# Autodesk Inventor assembly: Door Moulding Assembled
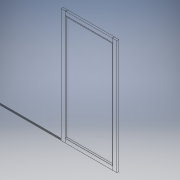
[picture p0: Inventor's stored thumbnail of the model, 180x180]
Saved by Autodesk Inventor 2016 (Build 200138000, 138)
## iProperties
Created: 2017-11-05
Part Number: Door Moulding Assembled
Document SubType Name: Assembly
Designer: mathaetaes
Author: mathaetaes
## Documents named in this file (4)
- E:\Projects\3D Printer\printer projects\My Designs\Bar Cabinet 2.20.2018\Door Moulding Assembled.iam
- E:\Projects\3D Printer\printer projects\My Designs\Bar Cabinet 2.20.2018\Cabinet Moulding Long.ipt
- E:\Projects\3D Printer\printer projects\My Designs\Bar Cabinet 2.20.2018\Door moulding slide-in panel.ipt
- E:\Projects\3D Printer\printer projects\My Designs\Bar Cabinet 2.20.2018\Cabinet Moulding Short.ipt
## Components (5 placed, 3 different names)
1. Cabinet Moulding Long:1 — Mate:2, Mate:3, Flush:2, Flush:4, Flush:5, Mate:6, Flush:6, Mate:7, Mate:8
2. Cabinet Moulding Long:2 — Mate:1, Mate:4, Flush:1, Flush:3
3. Door moulding slide-in panel:1 — Mate:5, Mate:6, Mate:7, Mate:8
4. Cabinet Moulding Short:1 — Mate:3, Flush:5, Flush:6
5. Cabinet Moulding Short:2 — Mate:1, Mate:2, Mate:4, Flush:1, Flush:2, Flush:3, Flush:4, Mate:5
## Relationships (14: Mate 8, Flush 6)
- Mate:1: Cabinet Moulding Long:2 ↔ Cabinet Moulding Short:2
- Mate:2: Cabinet Moulding Long:1 ↔ Cabinet Moulding Short:2
- Mate:3: Cabinet Moulding Long:1 ↔ Cabinet Moulding Short:1
- Mate:4: Cabinet Moulding Long:2 ↔ Cabinet Moulding Short:2
- Flush:1: Cabinet Moulding Long:2 ↔ Cabinet Moulding Short:2
- Flush:2: Cabinet Moulding Long:1 ↔ Cabinet Moulding Short:2
- Flush:3: Cabinet Moulding Long:2 ↔ Cabinet Moulding Short:2
- Flush:4: Cabinet Moulding Long:1 ↔ Cabinet Moulding Short:2
- Flush:5: Cabinet Moulding Long:1 ↔ Cabinet Moulding Short:1
- Mate:5: Door moulding slide-in panel:1 ↔ Cabinet Moulding Short:2
- Mate:6: Cabinet Moulding Long:1 ↔ Door moulding slide-in panel:1
- Flush:6: Cabinet Moulding Long:1 ↔ Cabinet Moulding Short:1
- Mate:7: Cabinet Moulding Long:1 ↔ Door moulding slide-in panel:1
- Mate:8: Cabinet Moulding Long:1 ↔ Door moulding slide-in panel:1
